# Autodesk Inventor assembly: Aquire assembly v1
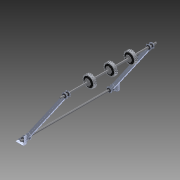
[picture p0: Inventor's stored thumbnail of the model, 180x180]
Saved by Autodesk Inventor 2014 SP1 (Build 180222100, 222)
## iProperties
Created: 2014-01-25
Part Number: Aquire assembly v1
Document SubType Name: Assembly
Designer: Paul
Author: Paul
## Documents named in this file (8)
- C:\FRC_CAD\4859cad\Robot\Actual Robot\Acquire\Aquire assembly v1.iam
- C:\FRC_CAD\4859cad\Robot\Actual Robot\Acquire\33 in hex shaft.ipt
- C:\FRC_CAD\4859cad\Robot\Actual Robot\Acquire\Corner Gusset.ipt
- C:\FRC_CAD\4859cad\Robot\Actual Robot\Acquire\End Cap Bearing Mount.ipt
- C:\FRC_CAD\4859cad\Robot\Actual Robot\Acquire\Hex bearing.ipt
- C:\FRC_CAD\4859cad\Robot\Actual Robot\Acquire\adjustable 1x1 tube.ipt
- C:\FRC_CAD\4859cad\Robot\Actual Robot\Acquire\4 in wheel.iam
- C:\FRC_CAD\4859cad\Robot\Actual Robot\Acquire\500EX Hex wheel Hub.ipt
## Components (30 placed, 7 different names)
1. 33 in hex shaft:1 — Mate:1, Mate:2, Mate:5, Mate:6, Mate:19, Mate:20, Mate:21, Mate:34
2. Corner Gusset:1 — Mate:4, Mate:8, Flush:2, Mate:35, Angle:1
3. Corner Gusset:2 — Mate:3, Flush:2, Mate:22, Mate:37
4. End Cap Bearing Mount:1 — Mate:9, Mate:10, Mate:11, Mate:15, Mate:16, Mate:22
5. End Cap Bearing Mount:2 — Mate:12, Mate:13, Mate:14, Mate:17, Mate:18, Rotation:1
6. Hex bearing:1 — Mate:17, Mate:18, Mate:19, Rotation:1
7. Hex bearing:2 — Mate:4, Mate:5, Mate:6, Mate:8, Mate:33
8. Hex bearing:3 — Mate:1, Mate:2, Mate:3, Mate:37
9. Hex bearing:4 — Mate:15, Mate:16, Mate:20, Mate:21
10. 33 in hex shaft:2 — Mate:48, Mate:49, Mate:50, Mate:51, Flush:9, Flush:10, Mate:52, Mate:53, Mate:54, Mate:55, Mate:92, Mate:93, Mate:95, Mate:96, Mate:100, Mate:101
11. adjustable 1x1 tube:1 — Mate:9, Mate:10, Mate:11, Mate:12, Mate:13, Mate:14, Flush:4, Mate:57, Mate:58, Mate:76, Mate:77, Mate:78
12. End Cap Bearing Mount:3
13. End Cap Bearing Mount:4 — Mate:35, Flush:11
14. Hex bearing:5 — Mate:33, Mate:34
15. Hex bearing:6
16. adjustable 1x1 tube:3 — Flush:4, Mate:46, Mate:47, Mate:79, Mate:80, Mate:81, Mate:82, Angle:1
17. End Cap Bearing Mount:5 — Mate:57, Mate:60, Mate:75, Mate:76, Mate:77
18. End Cap Bearing Mount:6 — Mate:56, Mate:58, Mate:59, Mate:78
19. End Cap Bearing Mount:7 — Mate:47, Flush:11, Mate:72, Mate:73, Mate:81, Mate:82
20. End Cap Bearing Mount:8 — Mate:46, Mate:61, Mate:74, Mate:79, Mate:80
21. Hex bearing:7 — Mate:54, Mate:55, Mate:60, Mate:75
22. Hex bearing:8 — Mate:50, Mate:51, Flush:9, Mate:72, Mate:73
23. Hex bearing:9 — Mate:48, Mate:49, Mate:61, Mate:74, Mate:102, Mate:103, Mate:104
24. Hex bearing:10 — Flush:10, Mate:52, Mate:53, Mate:56, Mate:59
25. 4 in wheel:4 [sub-assembly]
26. 500EX Hex wheel Hub:4 — Mate:92, Mate:93, Mate:103
27. 4 in wheel:5 [sub-assembly]
28. 500EX Hex wheel Hub:5 — Mate:95, Mate:96, Mate:102
29. 4 in wheel:6 [sub-assembly]
30. 500EX Hex wheel Hub:6 — Mate:100, Mate:101, Mate:104
## Relationships (87: Mate 80, Flush 5, RelateRotation 1, Angle 1)
- Mate:1: 33 in hex shaft:1 ↔ Hex bearing:3
- Mate:2: 33 in hex shaft:1 ↔ Hex bearing:3
- Mate:3: Corner Gusset:2 ↔ Hex bearing:3
- Mate:4: Corner Gusset:1 ↔ Hex bearing:2
- Mate:5: 33 in hex shaft:1 ↔ Hex bearing:2
- Mate:6: 33 in hex shaft:1 ↔ Hex bearing:2
- Mate:8: Corner Gusset:1 ↔ Hex bearing:2
- Flush:2: Corner Gusset:1 ↔ Corner Gusset:2
- Mate:9: End Cap Bearing Mount:1 ↔ adjustable 1x1 tube:1
- Mate:10: End Cap Bearing Mount:1 ↔ adjustable 1x1 tube:1
- Mate:11: End Cap Bearing Mount:1 ↔ adjustable 1x1 tube:1
- Mate:12: End Cap Bearing Mount:2 ↔ adjustable 1x1 tube:1
- Mate:13: End Cap Bearing Mount:2 ↔ adjustable 1x1 tube:1
- Mate:14: End Cap Bearing Mount:2 ↔ adjustable 1x1 tube:1
- Mate:15: End Cap Bearing Mount:1 ↔ Hex bearing:4
- Mate:16: End Cap Bearing Mount:1 ↔ Hex bearing:4
- Mate:17: End Cap Bearing Mount:2 ↔ Hex bearing:1
- Mate:18: End Cap Bearing Mount:2 ↔ Hex bearing:1
- Mate:19: 33 in hex shaft:1 ↔ Hex bearing:1
- Mate:20: 33 in hex shaft:1 ↔ Hex bearing:4
- Mate:21: 33 in hex shaft:1 ↔ Hex bearing:4
- Mate:22 (12.7 mm): Corner Gusset:2 ↔ End Cap Bearing Mount:1
- [Mate]: End Cap Bearing Mount:3 ↔ adjustable 1x1 tube:3
- [Mate]: End Cap Bearing Mount:3 ↔ adjustable 1x1 tube:3
- [Mate]: End Cap Bearing Mount:3 ↔ adjustable 1x1 tube:3
- [Mate]: End Cap Bearing Mount:4 ↔ adjustable 1x1 tube:3
- [Mate]: End Cap Bearing Mount:4 ↔ adjustable 1x1 tube:3
- [Mate]: End Cap Bearing Mount:4 ↔ adjustable 1x1 tube:3
- [Mate]: End Cap Bearing Mount:3 ↔ Hex bearing:6
- [Mate]: End Cap Bearing Mount:3 ↔ Hex bearing:6
- [Mate]: End Cap Bearing Mount:4 ↔ Hex bearing:5
- [Mate]: End Cap Bearing Mount:4 ↔ Hex bearing:5
- Mate:33: Hex bearing:2 ↔ Hex bearing:5
- Mate:34: 33 in hex shaft:1 ↔ Hex bearing:5
- Flush:4: adjustable 1x1 tube:1 ↔ adjustable 1x1 tube:3
- Rotation:1 [RelateRotation] (1 ul): End Cap Bearing Mount:2 ↔ Hex bearing:1
- Mate:35 (12.7 mm): Corner Gusset:1 ↔ End Cap Bearing Mount:4
- Mate:37: Corner Gusset:2 ↔ Hex bearing:3
- Mate:46: adjustable 1x1 tube:3 ↔ End Cap Bearing Mount:8
- Mate:47: adjustable 1x1 tube:3 ↔ End Cap Bearing Mount:7
- Mate:48: 33 in hex shaft:2 ↔ Hex bearing:9
- Mate:49: 33 in hex shaft:2 ↔ Hex bearing:9
- Mate:50: 33 in hex shaft:2 ↔ Hex bearing:8
- Mate:51: 33 in hex shaft:2 ↔ Hex bearing:8
- Flush:9 (34.925 mm): 33 in hex shaft:2 ↔ Hex bearing:8
- Flush:10 (34.925 mm): 33 in hex shaft:2 ↔ Hex bearing:10
- Mate:52: 33 in hex shaft:2 ↔ Hex bearing:10
- Mate:53: 33 in hex shaft:2 ↔ Hex bearing:10
- Mate:54: 33 in hex shaft:2 ↔ Hex bearing:7
- Mate:55: 33 in hex shaft:2 ↔ Hex bearing:7
- Mate:56: End Cap Bearing Mount:6 ↔ Hex bearing:10
- Mate:57: adjustable 1x1 tube:1 ↔ End Cap Bearing Mount:5
- Mate:58: adjustable 1x1 tube:1 ↔ End Cap Bearing Mount:6
- Mate:59: End Cap Bearing Mount:6 ↔ Hex bearing:10
- Mate:60: End Cap Bearing Mount:5 ↔ Hex bearing:7
- Mate:61: End Cap Bearing Mount:8 ↔ Hex bearing:9
- Flush:11: End Cap Bearing Mount:4 ↔ End Cap Bearing Mount:7
- Mate:72: End Cap Bearing Mount:7 ↔ Hex bearing:8
- Mate:73: End Cap Bearing Mount:7 ↔ Hex bearing:8
- Mate:74: End Cap Bearing Mount:8 ↔ Hex bearing:9
- Mate:75: End Cap Bearing Mount:5 ↔ Hex bearing:7
- Mate:76: adjustable 1x1 tube:1 ↔ End Cap Bearing Mount:5
- Mate:77: adjustable 1x1 tube:1 ↔ End Cap Bearing Mount:5
- Mate:78: adjustable 1x1 tube:1 ↔ End Cap Bearing Mount:6
- Mate:79: adjustable 1x1 tube:3 ↔ End Cap Bearing Mount:8
- Mate:80: adjustable 1x1 tube:3 ↔ End Cap Bearing Mount:8
- Mate:81: adjustable 1x1 tube:3 ↔ End Cap Bearing Mount:7
- Mate:82: adjustable 1x1 tube:3 ↔ End Cap Bearing Mount:7
- Angle:1 (55.19 deg): Corner Gusset:1 ↔ adjustable 1x1 tube:3
- [Mate]: 4 in wheel:4 ↔ 500EX Hex wheel Hub:4
- [Mate]: 4 in wheel:4 ↔ 500EX Hex wheel Hub:4
- [Mate]: 4 in wheel:4 ↔ 500EX Hex wheel Hub:4
- [Mate]: 4 in wheel:5 ↔ 500EX Hex wheel Hub:5
- [Mate]: 4 in wheel:5 ↔ 500EX Hex wheel Hub:5
- [Mate]: 4 in wheel:5 ↔ 500EX Hex wheel Hub:5
- Mate:92: 33 in hex shaft:2 ↔ 500EX Hex wheel Hub:4
- Mate:93: 33 in hex shaft:2 ↔ 500EX Hex wheel Hub:4
- Mate:95: 33 in hex shaft:2 ↔ 500EX Hex wheel Hub:5
- Mate:96: 33 in hex shaft:2 ↔ 500EX Hex wheel Hub:5
- [Mate]: 4 in wheel:6 ↔ 500EX Hex wheel Hub:6
- [Mate]: 4 in wheel:6 ↔ 500EX Hex wheel Hub:6
- [Mate]: 4 in wheel:6 ↔ 500EX Hex wheel Hub:6
- Mate:100: 33 in hex shaft:2 ↔ 500EX Hex wheel Hub:6
- Mate:101: 33 in hex shaft:2 ↔ 500EX Hex wheel Hub:6
- Mate:102 (164.592 mm): Hex bearing:9 ↔ 500EX Hex wheel Hub:5
- Mate:103 (347.8784 mm): Hex bearing:9 ↔ 500EX Hex wheel Hub:4
- Mate:104 (521.8176 mm): Hex bearing:9 ↔ 500EX Hex wheel Hub:6
## Named parameters: d27_d12 = 0 mm, d28_d13 = 0 mm, d29_d14 = 0 mm, d30_d15 = 0 mm, d31_d16 = 0 mm, d32_d17 = 0 mm, d33_d19 = 0 mm, d34_d20 = 0 mm, d35_d21 = 0 mm, d36_d22 = 0 mm, d110_d107 = 0 mm, d111_d108 = 0 mm, d112_d109 = 0 mm, d113_d107 = 0 mm, d114_d108 = 0 mm, d115_d109 = 0 mm, d121_d110_d107 = 0 mm, d122_d111_d108 = 0 mm, d123_d112_d109 = 0 mm
